# Autodesk Inventor assembly: 673
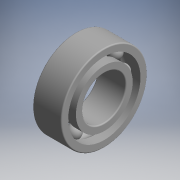
[picture p0: Inventor's stored thumbnail of the model, 180x180]
Saved by Autodesk Inventor 2017.3 (Build 213256000, 256)
## iProperties
Category: PARTsolutions
Company: NTN
Part Number: 673
Catalog Web Link: www.cadenas.de
Description: Open type-
Vendor: NTN
Document SubType Name: Assembly
Designer: partserver
Manufacturer: NTN
Mass: 0.0279443 g
Surface Area: 1.6369 cm^2
Volume: 0.0279443 cm^3
Density: 1 g/cm^3
Title: 673
Author: Cadenas PARTsolutions
PSOL_IDENT_0: {$CADENAS_DATA\23d-libs\ntn\ball_roller_bearings\miniature_extra_small_bb\metric_system_sizes\mss_ot
PSOL_IDENT_1: _asmtab.prj},164 {VTYP=3D},{STYP=ASSTAB},{NB=673},{LINA=673},{NN=Open type},{DATE=21.12.2021 04:23:0
PSOL_IDENT_2: 5},{GEOMDATE=10.03.2020 01:12:04},{VERSION=},{LINEID=450},{WBVAR=},{WBNUMERIC=}  {NB=673},{LINA=673}
PSOL_IDENT_3: ,{KT=DUMMY},{IDNR=},{SD=3.0},{D=6},{B=2.0},{B1=2.5},{D1=7.2},{D2=7.2},{C1=0.6},{C2=0.6},{R=0.08},{OR
PSOL_IDENT_4: DER=673},{CR=268},{COR=94},{CU=2.47},{CRF=25},{CORF=9,5},{LSG=60 000},{LSO=71 000},{MASS=0.20},{ORDE
PSOL_IDENT_5: R1=673},{WSS=WA673SA},{WDS=SSA},{UTWF=FL673},{FORSS=FLWA673SA},{FORDS=SSA},{DA1=3,6},{DA2=4,1},{DA=5
PSOL_IDENT_6: ,4},{RAS=0,08},{MASS1=0.26},{VERS=1},{X=1.5},{N=9},{O=14.13},{RB=0.444},{PPATH=mss_asmtpl.prj}
NB: 673
NN: Open type
NBSYN: $ORDER.
LINA: 673
CATALOG: NTN Corporation
SD: 3
D: 6
B: 2
R: 0.08
ORDER: 673
CR: 268
COR: 94
CU: 2.47
LSG: 60 000
LSO: 71 000
MASS: 0.2
SUPPLIER: NTN
ARTICLENO: 673
BOMINFO: 673
CREATOR: CADENAS GmbH
## Documents named in this file (4)
- e:\temp\worker_40\temp\exporttempdir_3080_331_G1Pk3\format_0\673.iam
- e:\temp\worker_40\temp\exporttempdir_3080_331_G1Pk3\format_0\673 Inner ring.ipt
- e:\temp\worker_40\temp\exporttempdir_3080_331_G1Pk3\format_0\673 Outer ring.ipt
- e:\temp\worker_40\temp\exporttempdir_3080_331_G1Pk3\format_0\673 Ball.ipt
## Components (11 placed, 3 different names)
1. 673 Inner ring:1 — mss_ir_Z@1 <-> mss_or_Z@2
2. 673 Outer ring:1 — mss_ir_Z@1 <-> mss_or_Z@2, mss_or2_1_XY@2 <-> mss_ball_XY@3, mss_or2_1_Z@2 <-> mss_ball_Z@3, mss_or2_1_YZ@2 <-> mss_ball_YZ@3, mss_or2_2_XY@2 <-> mss_ball_XY@4, mss_or2_2_Z@2 <-> mss_ball_Z@4, mss_or2_2_YZ@2 <-> mss_ball_YZ@4, mss_or2_3_XY@2 <-> mss_ball_XY@5, mss_or2_3_Z@2 <-> mss_ball_Z@5, mss_or2_3_YZ@2 <-> mss_ball_YZ@5, mss_or2_4_XY@2 <-> mss_ball_XY@6, mss_or2_4_Z@2 <-> mss_ball_Z@6, mss_or2_4_YZ@2 <-> mss_ball_YZ@6, mss_or2_5_XY@2 <-> mss_ball_XY@7, mss_or2_5_Z@2 <-> mss_ball_Z@7, mss_or2_5_YZ@2 <-> mss_ball_YZ@7, mss_or2_6_XY@2 <-> mss_ball_XY@8, mss_or2_6_Z@2 <-> mss_ball_Z@8, mss_or2_6_YZ@2 <-> mss_ball_YZ@8, mss_or2_7_XY@2 <-> mss_ball_XY@9, mss_or2_7_Z@2 <-> mss_ball_Z@9, mss_or2_7_YZ@2 <-> mss_ball_YZ@9, mss_or2_8_XY@2 <-> mss_ball_XY@10, mss_or2_8_Z@2 <-> mss_ball_Z@10, mss_or2_8_YZ@2 <-> mss_ball_YZ@10, mss_or2_9_XY@2 <-> mss_ball_XY@11, mss_or2_9_Z@2 <-> mss_ball_Z@11, mss_or2_9_YZ@2 <-> mss_ball_YZ@11
3. 673 Ball:1 — mss_or2_1_XY@2 <-> mss_ball_XY@3, mss_or2_1_Z@2 <-> mss_ball_Z@3, mss_or2_1_YZ@2 <-> mss_ball_YZ@3
4. 673 Ball:2 — mss_or2_2_XY@2 <-> mss_ball_XY@4, mss_or2_2_Z@2 <-> mss_ball_Z@4, mss_or2_2_YZ@2 <-> mss_ball_YZ@4
5. 673 Ball:3 — mss_or2_3_XY@2 <-> mss_ball_XY@5, mss_or2_3_Z@2 <-> mss_ball_Z@5, mss_or2_3_YZ@2 <-> mss_ball_YZ@5
6. 673 Ball:4 — mss_or2_4_XY@2 <-> mss_ball_XY@6, mss_or2_4_Z@2 <-> mss_ball_Z@6, mss_or2_4_YZ@2 <-> mss_ball_YZ@6
7. 673 Ball:5 — mss_or2_5_XY@2 <-> mss_ball_XY@7, mss_or2_5_Z@2 <-> mss_ball_Z@7, mss_or2_5_YZ@2 <-> mss_ball_YZ@7
8. 673 Ball:6 — mss_or2_6_XY@2 <-> mss_ball_XY@8, mss_or2_6_Z@2 <-> mss_ball_Z@8, mss_or2_6_YZ@2 <-> mss_ball_YZ@8
9. 673 Ball:7 — mss_or2_7_XY@2 <-> mss_ball_XY@9, mss_or2_7_Z@2 <-> mss_ball_Z@9, mss_or2_7_YZ@2 <-> mss_ball_YZ@9
10. 673 Ball:8 — mss_or2_8_XY@2 <-> mss_ball_XY@10, mss_or2_8_Z@2 <-> mss_ball_Z@10, mss_or2_8_YZ@2 <-> mss_ball_YZ@10
11. 673 Ball:9 — mss_or2_9_XY@2 <-> mss_ball_XY@11, mss_or2_9_Z@2 <-> mss_ball_Z@11, mss_or2_9_YZ@2 <-> mss_ball_YZ@11
## Relationships (28: Mate 19, Angle 9)
- mss_ir_Z@1 <-> mss_or_Z@2 [Mate]: 673 Inner ring:1 ↔ 673 Outer ring:1
- mss_or2_1_XY@2 <-> mss_ball_XY@3 [Mate]: 673 Outer ring:1 ↔ 673 Ball:1
- mss_or2_1_Z@2 <-> mss_ball_Z@3 [Mate]: 673 Outer ring:1 ↔ 673 Ball:1
- mss_or2_1_YZ@2 <-> mss_ball_YZ@3 [Angle] (0 deg): 673 Outer ring:1 ↔ 673 Ball:1
- mss_or2_2_XY@2 <-> mss_ball_XY@4 [Mate]: 673 Outer ring:1 ↔ 673 Ball:2
- mss_or2_2_Z@2 <-> mss_ball_Z@4 [Mate]: 673 Outer ring:1 ↔ 673 Ball:2
- mss_or2_2_YZ@2 <-> mss_ball_YZ@4 [Angle] (0 deg): 673 Outer ring:1 ↔ 673 Ball:2
- mss_or2_3_XY@2 <-> mss_ball_XY@5 [Mate]: 673 Outer ring:1 ↔ 673 Ball:3
- mss_or2_3_Z@2 <-> mss_ball_Z@5 [Mate]: 673 Outer ring:1 ↔ 673 Ball:3
- mss_or2_3_YZ@2 <-> mss_ball_YZ@5 [Angle] (0 deg): 673 Outer ring:1 ↔ 673 Ball:3
- mss_or2_4_XY@2 <-> mss_ball_XY@6 [Mate]: 673 Outer ring:1 ↔ 673 Ball:4
- mss_or2_4_Z@2 <-> mss_ball_Z@6 [Mate]: 673 Outer ring:1 ↔ 673 Ball:4
- mss_or2_4_YZ@2 <-> mss_ball_YZ@6 [Angle] (0 deg): 673 Outer ring:1 ↔ 673 Ball:4
- mss_or2_5_XY@2 <-> mss_ball_XY@7 [Mate]: 673 Outer ring:1 ↔ 673 Ball:5
- mss_or2_5_Z@2 <-> mss_ball_Z@7 [Mate]: 673 Outer ring:1 ↔ 673 Ball:5
- mss_or2_5_YZ@2 <-> mss_ball_YZ@7 [Angle] (0 deg): 673 Outer ring:1 ↔ 673 Ball:5
- mss_or2_6_XY@2 <-> mss_ball_XY@8 [Mate]: 673 Outer ring:1 ↔ 673 Ball:6
- mss_or2_6_Z@2 <-> mss_ball_Z@8 [Mate]: 673 Outer ring:1 ↔ 673 Ball:6
- mss_or2_6_YZ@2 <-> mss_ball_YZ@8 [Angle] (0 deg): 673 Outer ring:1 ↔ 673 Ball:6
- mss_or2_7_XY@2 <-> mss_ball_XY@9 [Mate]: 673 Outer ring:1 ↔ 673 Ball:7
- mss_or2_7_Z@2 <-> mss_ball_Z@9 [Mate]: 673 Outer ring:1 ↔ 673 Ball:7
- mss_or2_7_YZ@2 <-> mss_ball_YZ@9 [Angle] (0 deg): 673 Outer ring:1 ↔ 673 Ball:7
- mss_or2_8_XY@2 <-> mss_ball_XY@10 [Mate]: 673 Outer ring:1 ↔ 673 Ball:8
- mss_or2_8_Z@2 <-> mss_ball_Z@10 [Mate]: 673 Outer ring:1 ↔ 673 Ball:8
- mss_or2_8_YZ@2 <-> mss_ball_YZ@10 [Angle] (0 deg): 673 Outer ring:1 ↔ 673 Ball:8
- mss_or2_9_XY@2 <-> mss_ball_XY@11 [Mate]: 673 Outer ring:1 ↔ 673 Ball:9
- mss_or2_9_Z@2 <-> mss_ball_Z@11 [Mate]: 673 Outer ring:1 ↔ 673 Ball:9
- mss_or2_9_YZ@2 <-> mss_ball_YZ@11 [Angle] (0 deg): 673 Outer ring:1 ↔ 673 Ball:9
